# Autodesk Inventor assembly: Fender and Igus
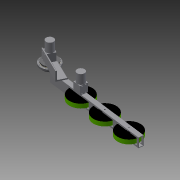
[picture p0: Inventor's stored thumbnail of the model, 180x180]
Saved by Autodesk Inventor 2015 (Build 190159000, 159)
## iProperties
Created: 2015-01-19
Part Number: Fender and Igus
Document SubType Name: Assembly
Designer: chapale16
Author: chapale16
## Documents named in this file (3)
- \\lhssvr02\Homedirs\Robotics Club\CAD Model 2015\Fender and Igus.iam
- \\lhssvr02\Homedirs\Robotics Club\CAD Model 2015\Igus and Arm Bracket.iam
- \\lhssvr02\Homedirs\Robotics Club\CAD Model 2015\Game Components\The Tote Collector-Arms\Collector Arms v2.0_MIR_MIR.iam
## Components (2 placed, 2 different names)
1. Igus and Arm Bracket:1 [sub-assembly] — Mate:1
2. Collector Arms v2.0_MIR_MIR:1 [sub-assembly] — Mate:1
## Relationships (1: Mate 1)
- Mate:1: Igus and Arm Bracket:1 ↔ Collector Arms v2.0_MIR_MIR:1
